# Autodesk Inventor assembly: GreyT Telescope All
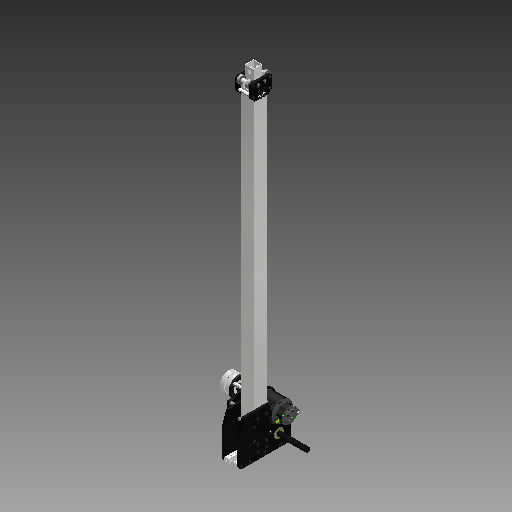
[picture p0: Inventor's stored thumbnail of the model, 512x512]
Saved by Autodesk Inventor 2022 (Build 260153000, 153)
## iProperties
Created: 2021-11-19
Part Number: GreyT Telescope All
Description: STEP AP214
Document SubType Name: Assembly
Sending System: SolidWorks 2020
Preprocessor: SwSTEP 2.0
Title: WCP - Greyt Telescope (Stages #1-4).step
Revision Number: ANY
## Documents named in this file (5)
- C:\Users\Cal\Desktop\Robotics\Design\Collaborative\Collaborative Parts Library\Elevators\GreyT Telescope\GreyT Telescope All.iam
- C:\Users\Cal\Desktop\Robotics\Design\Collaborative\Collaborative Parts Library\Elevators\GreyT Telescope\GreyT Telescope Top Block.iam
- C:\Users\Cal\Desktop\Robotics\Design\Collaborative\Collaborative Parts Library\Elevators\GreyT Telescope\GreyT Telescope Bottom Block.iam
- C:\Users\Cal\Desktop\Robotics\Design\Collaborative\Collaborative Parts Library\Elevators\GreyT Telescope\GreyT Telescope Gearbox.iam
- C:\Users\Cal\Desktop\Robotics\Design\Collaborative\Collaborative Parts Library\Elevators\GreyT Telescope\GreyT Tube Template.ipt
## Components (5 placed, 4 different names)
1. GreyT Telescope Top Block:1 [sub-assembly] — Insert:2, Angle:2, Tangent:2
2. GreyT Telescope Gearbox:1 [sub-assembly] — Insert:1, Angle:1, Tangent:1
3. GreyT Tube Template:1 — Insert:1, Angle:1, Insert:2, Angle:2, Flush:1, Flush:2
4. GreyT Tube Template:2 — Mate:1, Mate:2, Mate:3, Flush:1, Flush:2
5. GreyT Telescope Bottom Block:1 [sub-assembly] — Mate:1, Mate:2, Mate:3, Tangent:1, Tangent:2
## Relationships (11: Mate 3, Insert 2, Angle 2, Flush 2, Tangent 2)
- Insert:1: GreyT Telescope Gearbox:1 ↔ GreyT Tube Template:1
- Angle:1 (0 deg): GreyT Telescope Gearbox:1 ↔ GreyT Tube Template:1
- Insert:2: GreyT Telescope Top Block:1 ↔ GreyT Tube Template:1
- Angle:2 (0 deg): GreyT Telescope Top Block:1 ↔ GreyT Tube Template:1
- Mate:1: GreyT Tube Template:2 ↔ GreyT Telescope Bottom Block:1
- Mate:2: GreyT Tube Template:2 ↔ GreyT Telescope Bottom Block:1
- Mate:3: GreyT Tube Template:2 ↔ GreyT Telescope Bottom Block:1
- Flush:1: GreyT Tube Template:1 ↔ GreyT Tube Template:2
- Flush:2: GreyT Tube Template:1 ↔ GreyT Tube Template:2
- Tangent:1: GreyT Telescope Gearbox:1 ↔ GreyT Telescope Bottom Block:1
- Tangent:2: GreyT Telescope Top Block:1 ↔ GreyT Telescope Bottom Block:1
